# Autodesk Inventor assembly: Backpack
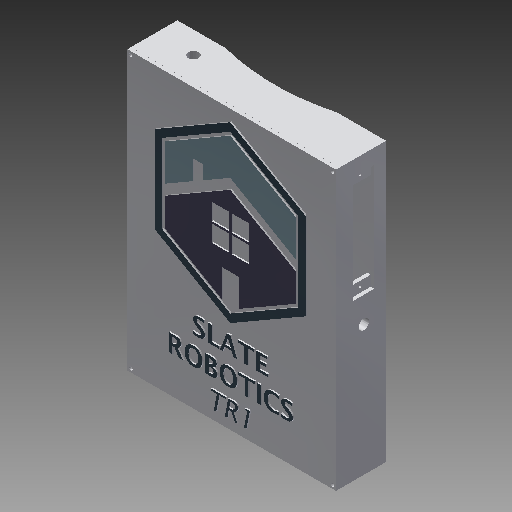
[picture p0: Inventor's stored thumbnail of the model, 512x512]
Saved by Autodesk Inventor 2017 SP1 (Build 210196100, 196)
## iProperties
Created: 2017-09-05
Part Number: Backpack
Document SubType Name: Assembly
Designer: Zach
Author: Zach
## Documents named in this file (5)
- C:\Users\Zach\Documents\GitHub\tr1\src\Body\Chest Assembly\Backpack Assembly\Backpack.iam
- C:\Users\Zach\Documents\GitHub\tr1\src\Body\Chest Assembly\Backpack Assembly\BP001b.ipt
- C:\Users\Zach\Documents\GitHub\tr1\src\Body\Chest Assembly\Backpack Assembly\BP002b.ipt
- C:\Users\Zach\Documents\GitHub\tr1\src\Body\Chest Assembly\Backpack Assembly\BP003.ipt
- C:\Users\Zach\Documents\GitHub\tr1\src\Body\Chest Assembly\Backpack Assembly\BP004.ipt
## Components (4 placed, 4 different names)
1. BP001b:1 — Mate:1, Mate:2, Mate:3, Mate:4, Mate:5, Mate:6, Mate:7
2. BP002b:1 — Mate:1, Mate:2, Mate:3
3. BP003:1 — Mate:4
4. BP004:1 — Mate:5, Mate:6, Mate:7
## Relationships (7: Mate 7)
- Mate:1: BP001b:1 ↔ BP002b:1
- Mate:2: BP001b:1 ↔ BP002b:1
- Mate:3: BP001b:1 ↔ BP002b:1
- Mate:4: BP001b:1 ↔ BP003:1
- Mate:5: BP001b:1 ↔ BP004:1
- Mate:6: BP001b:1 ↔ BP004:1
- Mate:7: BP001b:1 ↔ BP004:1
